# Autodesk Inventor assembly: X-Gantry Joiner Left Assembly
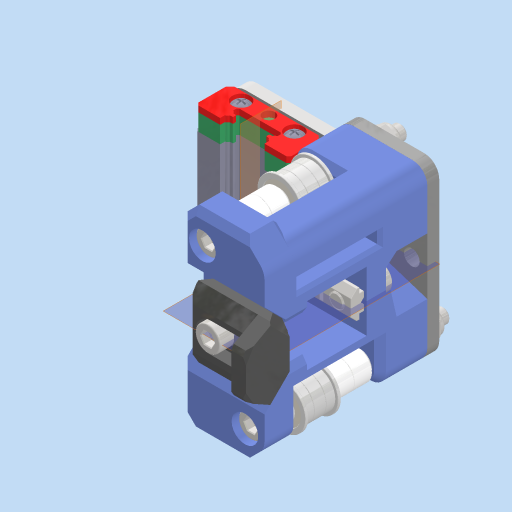
[picture p0: Inventor's stored thumbnail of the model, 512x512]
Saved by Autodesk Inventor 2023.2 (Build 272271000, 271)
## iProperties
Created: 2023-11-28
Part Number: X-Gantry Joiner Left Assembly
Document SubType Name: Assembly
Designer: Nils Bade
Author: Nils Bade
## Documents named in this file (15)
- C:\Users\nilsb\Documents\Inventor\Projektarbeit-Bade\RatRig_Bade\X-Gantry Joiner Left Assembly.iam
- C:\Users\nilsb\Documents\Inventor\Projektarbeit-Bade\RatRig_modified\XY Joiner Plate for 4040.ipt
- C:\Users\nilsb\Documents\Inventor\Projektarbeit-Bade\RatRig_modified\MGN15 Linear-Rail-Block.ipt
- C:\Users\nilsb\Documents\Inventor\Projektarbeit-Bade\Schrauben\Cap Head Screw M3x12 v2.ipt
- C:\Users\nilsb\Documents\Inventor\Projektarbeit-Bade\RatRig_Standards\T-Nut - Square type for 2020 - M5 v2.ipt
- C:\Users\nilsb\Documents\Inventor\Projektarbeit-Bade\Schrauben\Cap Head Screw M5x10 v2.ipt
- C:\Users\nilsb\Documents\Inventor\Projektarbeit-Bade\RatRig_Standards\x_endstop_block_3.1 v2.ipt
- C:\Users\nilsb\Documents\Inventor\Projektarbeit-Bade\Schrauben\Cap Head Screw M5x18 v2.ipt
- C:\Users\nilsb\Documents\Inventor\Projektarbeit-Bade\Schrauben\Cap Head Screw M5x60.ipt
- C:\Users\nilsb\Documents\Inventor\Projektarbeit-Bade\RatRig_Standards\Hex Locking Nut - M5 v2.ipt
- C:\Users\nilsb\Documents\Inventor\Projektarbeit-Bade\RatRig_Standards\Mini Precision Shim - 8x5x1mm v2.ipt
- C:\Users\nilsb\Documents\Inventor\Projektarbeit-Bade\RatRig_Standards\Ball Bearing - F695ZZ v1.ipt
- C:\Users\nilsb\Documents\Inventor\Projektarbeit-Bade\RatRig_Standards\Ball Bearing - 695ZZ v1.ipt
- C:\Users\nilsb\Documents\Inventor\Projektarbeit-Bade\RatRig_Standards\Aluminium Spacer - 6mm v2.ipt
- C:\Users\nilsb\Documents\Inventor\Projektarbeit-Bade\RatRig_modified\xy Joiner Left for 4040 V1.ipt
## Components (34 placed, 14 different names)
1. xy Joiner Left for 4040 V1:2
2. xy Joiner Plate for 4040:1 — Passend:4, Passend:5, Passend:6, Passend:7, Passend:8, Passend:9, Passend:10, Passend:11, Passend:12, Passend:13, Passend:14, Passend:35, Passend:36
3. MGN15 Linear-Rail-Block:1 — Passend:4, Passend:5, Passend:6
4. Cap Head Screw M3x12 v2:1 — Passend:7, Passend:14
5. Cap Head Screw M3x12 v2:2 — Passend:9, Passend:13
6. Cap Head Screw M3x12 v2:3 — Passend:10, Passend:11
7. Cap Head Screw M3x12 v2:4 — Passend:8, Passend:12
8. T-Nut - Square type for 2020 - M5 v2:1
9. T-Nut - Square type for 2020 - M5 v2:3
10. T-Nut - Square type for 2020 - M5 v2:4
11. Cap Head Screw M5x10 v2:1
12. Cap Head Screw M5x10 v2:2
13. x_endstop_block_3.1 v2:1 — Passend:27, Passend:28
14. Cap Head Screw M5x18 v2:1 — Passend:27, Passend:28
15. Cap Head Screw M5x60:1 — Passend:33, Passend:53, Passend:55, Passend:57, Passend:59, Passend:61, Passend:63, Passend:65, Passend:67
16. Cap Head Screw M5x60:2 — Passend:34, Passend:37, Passend:39, Passend:41, Passend:43, Passend:45, Passend:47, Passend:49, Passend:51
17. Hex Locking Nut - M5 v2:1 — Passend:33, Passend:36
18. Hex Locking Nut - M5 v2:2 — Passend:34, Passend:35
19. Mini Precision Shim - 8x5x1mm v2:1 — Passend:51, Passend:52
20. Mini Precision Shim - 8x5x1mm v2:2 — Passend:45, Passend:46, Passend:48
21. Mini Precision Shim - 8x5x1mm v2:3 — Passend:37, Passend:40
22. Mini Precision Shim - 8x5x1mm v2:4 — Passend:53, Passend:56
23. Mini Precision Shim - 8x5x1mm v2:5 — Passend:61, Passend:62, Passend:64
24. Mini Precision Shim - 8x5x1mm v2:6 — Passend:67, Passend:68
25. Ball Bearing - F695ZZ v1:1 — Passend:43, Passend:44, Passend:46
26. Ball Bearing - F695ZZ v1:2 — Passend:55, Passend:56, Passend:58
27. Ball Bearing - F695ZZ v1:3 — Passend:59, Passend:60, Passend:62
28. Ball Bearing - F695ZZ v1:4 — Passend:39, Passend:40, Passend:42
29. Ball Bearing - 695ZZ v1:1 — Passend:41, Passend:42, Passend:44
30. Ball Bearing - 695ZZ v1:2 — Passend:57, Passend:58, Passend:60
31. Aluminium Spacer - 6mm v2:1 — Passend:47, Passend:48, Passend:50
32. Aluminium Spacer - 6mm v2:2 — Passend:49, Passend:50, Passend:52
33. Aluminium Spacer - 6mm v2:3 — Passend:63, Passend:64, Passend:66
34. Aluminium Spacer - 6mm v2:4 — Passend:65, Passend:66, Passend:68
## Relationships (72: Mate 68, Angle 4)
- [Mate]: xy Joiner Left for 4040 V1:2 ↔ xy Joiner Plate for 4040:1
- [Mate]: xy Joiner Left for 4040 V1:2 ↔ xy Joiner Plate for 4040:1
- [Mate]: xy Joiner Left for 4040 V1:2 ↔ xy Joiner Plate for 4040:1
- Passend:4 [Mate]: xy Joiner Plate for 4040:1 ↔ MGN15 Linear-Rail-Block:1
- Passend:5 [Mate]: xy Joiner Plate for 4040:1 ↔ MGN15 Linear-Rail-Block:1
- Passend:6 [Mate]: xy Joiner Plate for 4040:1 ↔ MGN15 Linear-Rail-Block:1
- Passend:7 [Mate]: xy Joiner Plate for 4040:1 ↔ Cap Head Screw M3x12 v2:1
- Passend:8 [Mate]: xy Joiner Plate for 4040:1 ↔ Cap Head Screw M3x12 v2:4
- Passend:9 [Mate]: xy Joiner Plate for 4040:1 ↔ Cap Head Screw M3x12 v2:2
- Passend:10 [Mate]: xy Joiner Plate for 4040:1 ↔ Cap Head Screw M3x12 v2:3
- Passend:11 [Mate]: xy Joiner Plate for 4040:1 ↔ Cap Head Screw M3x12 v2:3
- Passend:12 [Mate]: xy Joiner Plate for 4040:1 ↔ Cap Head Screw M3x12 v2:4
- Passend:13 [Mate]: xy Joiner Plate for 4040:1 ↔ Cap Head Screw M3x12 v2:2
- Passend:14 [Mate]: xy Joiner Plate for 4040:1 ↔ Cap Head Screw M3x12 v2:1
- [Mate]: xy Joiner Left for 4040 V1:2 ↔ T-Nut - Square type for 2020 - M5 v2:1
- [Mate]: xy Joiner Left for 4040 V1:2 ↔ T-Nut - Square type for 2020 - M5 v2:3
- [Mate]: xy Joiner Left for 4040 V1:2 ↔ T-Nut - Square type for 2020 - M5 v2:4
- [Angle] (0 deg): xy Joiner Left for 4040 V1:2 ↔ T-Nut - Square type for 2020 - M5 v2:1
- [Angle] (0 deg): xy Joiner Left for 4040 V1:2 ↔ T-Nut - Square type for 2020 - M5 v2:4
- [Angle] (0 deg): xy Joiner Left for 4040 V1:2 ↔ T-Nut - Square type for 2020 - M5 v2:3
- [Mate] (1.8 mm): xy Joiner Left for 4040 V1:2 ↔ T-Nut - Square type for 2020 - M5 v2:4
- [Mate] (1.8 mm): xy Joiner Left for 4040 V1:2 ↔ T-Nut - Square type for 2020 - M5 v2:3
- [Mate] (1.8 mm): xy Joiner Left for 4040 V1:2 ↔ T-Nut - Square type for 2020 - M5 v2:1
- [Mate]: xy Joiner Left for 4040 V1:2 ↔ Cap Head Screw M5x10 v2:1
- [Mate]: xy Joiner Left for 4040 V1:2 ↔ Cap Head Screw M5x10 v2:1
- [Mate]: xy Joiner Left for 4040 V1:2 ↔ Cap Head Screw M5x10 v2:2
- [Mate]: xy Joiner Left for 4040 V1:2 ↔ Cap Head Screw M5x10 v2:2
- [Mate]: xy Joiner Left for 4040 V1:2 ↔ x_endstop_block_3.1 v2:1
- [Angle] (0 deg): xy Joiner Left for 4040 V1:2 ↔ x_endstop_block_3.1 v2:1
- [Mate]: xy Joiner Left for 4040 V1:2 ↔ x_endstop_block_3.1 v2:1
- Passend:27 [Mate]: x_endstop_block_3.1 v2:1 ↔ Cap Head Screw M5x18 v2:1
- Passend:28 [Mate]: x_endstop_block_3.1 v2:1 ↔ Cap Head Screw M5x18 v2:1
- [Mate]: xy Joiner Left for 4040 V1:2 ↔ Cap Head Screw M5x60:1
- [Mate]: xy Joiner Left for 4040 V1:2 ↔ Cap Head Screw M5x60:2
- [Mate]: xy Joiner Left for 4040 V1:2 ↔ Cap Head Screw M5x60:2
- [Mate]: xy Joiner Left for 4040 V1:2 ↔ Cap Head Screw M5x60:1
- Passend:33 [Mate]: Cap Head Screw M5x60:1 ↔ Hex Locking Nut - M5 v2:1
- Passend:34 [Mate]: Cap Head Screw M5x60:2 ↔ Hex Locking Nut - M5 v2:2
- Passend:35 [Mate]: xy Joiner Plate for 4040:1 ↔ Hex Locking Nut - M5 v2:2
- Passend:36 [Mate]: xy Joiner Plate for 4040:1 ↔ Hex Locking Nut - M5 v2:1
- Passend:37 [Mate]: Cap Head Screw M5x60:2 ↔ Mini Precision Shim - 8x5x1mm v2:3
- Passend:39 [Mate]: Cap Head Screw M5x60:2 ↔ Ball Bearing - F695ZZ v1:4
- Passend:40 [Mate]: Mini Precision Shim - 8x5x1mm v2:3 ↔ Ball Bearing - F695ZZ v1:4
- Passend:41 [Mate]: Cap Head Screw M5x60:2 ↔ Ball Bearing - 695ZZ v1:1
- Passend:42 [Mate]: Ball Bearing - F695ZZ v1:4 ↔ Ball Bearing - 695ZZ v1:1
- Passend:43 [Mate]: Cap Head Screw M5x60:2 ↔ Ball Bearing - F695ZZ v1:1
- Passend:44 [Mate]: Ball Bearing - F695ZZ v1:1 ↔ Ball Bearing - 695ZZ v1:1
- Passend:45 [Mate]: Cap Head Screw M5x60:2 ↔ Mini Precision Shim - 8x5x1mm v2:2
- Passend:46 [Mate]: Mini Precision Shim - 8x5x1mm v2:2 ↔ Ball Bearing - F695ZZ v1:1
- Passend:47 [Mate]: Cap Head Screw M5x60:2 ↔ Aluminium Spacer - 6mm v2:1
- Passend:48 [Mate]: Mini Precision Shim - 8x5x1mm v2:2 ↔ Aluminium Spacer - 6mm v2:1
- Passend:49 [Mate]: Cap Head Screw M5x60:2 ↔ Aluminium Spacer - 6mm v2:2
- Passend:50 [Mate]: Aluminium Spacer - 6mm v2:1 ↔ Aluminium Spacer - 6mm v2:2
- Passend:51 [Mate]: Cap Head Screw M5x60:2 ↔ Mini Precision Shim - 8x5x1mm v2:1
- Passend:52 [Mate]: Mini Precision Shim - 8x5x1mm v2:1 ↔ Aluminium Spacer - 6mm v2:2
- Passend:53 [Mate]: Cap Head Screw M5x60:1 ↔ Mini Precision Shim - 8x5x1mm v2:4
- [Mate]: xy Joiner Left for 4040 V1:2 ↔ Mini Precision Shim - 8x5x1mm v2:4
- Passend:55 [Mate]: Cap Head Screw M5x60:1 ↔ Ball Bearing - F695ZZ v1:2
- Passend:56 [Mate]: Mini Precision Shim - 8x5x1mm v2:4 ↔ Ball Bearing - F695ZZ v1:2
- Passend:57 [Mate]: Cap Head Screw M5x60:1 ↔ Ball Bearing - 695ZZ v1:2
- Passend:58 [Mate]: Ball Bearing - F695ZZ v1:2 ↔ Ball Bearing - 695ZZ v1:2
- Passend:59 [Mate]: Cap Head Screw M5x60:1 ↔ Ball Bearing - F695ZZ v1:3
- Passend:60 [Mate]: Ball Bearing - F695ZZ v1:3 ↔ Ball Bearing - 695ZZ v1:2
- Passend:61 [Mate]: Cap Head Screw M5x60:1 ↔ Mini Precision Shim - 8x5x1mm v2:5
- Passend:62 [Mate]: Mini Precision Shim - 8x5x1mm v2:5 ↔ Ball Bearing - F695ZZ v1:3
- Passend:63 [Mate]: Cap Head Screw M5x60:1 ↔ Aluminium Spacer - 6mm v2:3
- Passend:64 [Mate]: Mini Precision Shim - 8x5x1mm v2:5 ↔ Aluminium Spacer - 6mm v2:3
- Passend:65 [Mate]: Cap Head Screw M5x60:1 ↔ Aluminium Spacer - 6mm v2:4
- Passend:66 [Mate]: Aluminium Spacer - 6mm v2:3 ↔ Aluminium Spacer - 6mm v2:4
- Passend:67 [Mate]: Cap Head Screw M5x60:1 ↔ Mini Precision Shim - 8x5x1mm v2:6
- Passend:68 [Mate]: Mini Precision Shim - 8x5x1mm v2:6 ↔ Aluminium Spacer - 6mm v2:4
- [Mate]: xy Joiner Left for 4040 V1:2 ↔ Mini Precision Shim - 8x5x1mm v2:1
